# Autodesk Inventor assembly: !Ramp
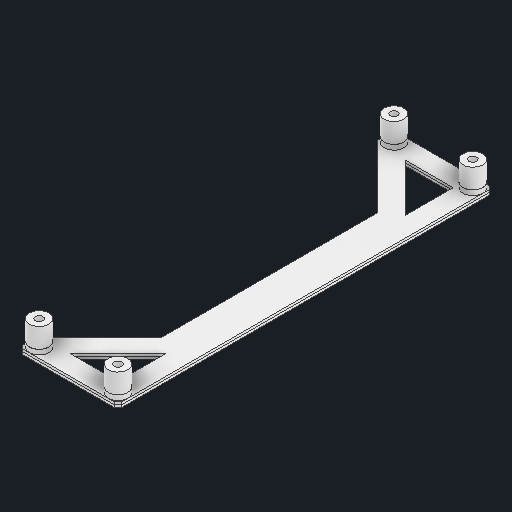
[picture p0: Inventor's stored thumbnail of the model, 512x512]
Saved by Autodesk Inventor 2025 (Build 290162000, 162)
## iProperties
Created: 2024-12-22
Part Number: !Ramp
Document SubType Name: Assembly
Designer: Averey Ku
Author: Averey Ku
## Documents named in this file (5)
- D:\VEX\High Stakes\CAD\V4\Chassis\Ramp\!Ramp.iam
- D:\VEX\High Stakes\CAD\V4\Chassis\Ramp\Custom Parts\Ramp.ipt
- D:\VEX\High Stakes\CAD\ROBOPROS-CAD-Inventor\Motion\Spacers\Spacer Nylon .500 OD.ipt
- D:\VEX\High Stakes\CAD\ROBOPROS-CAD-Inventor\Motion\Spacers\Spacer Nylon .500 OD\NSpacer White .500 OD x .500.ipt
- D:\VEX\High Stakes\CAD\ROBOPROS-CAD-Inventor\Motion\Spacers\Spacer Nylon .500 OD\NSpacer White .500 OD x .125.ipt
## Components (10 placed, 3 different names)
1. Ramp:1 — Insert:3, Insert:5, Insert:7, Insert:8, Insert:11, Mate:1
2. NSpacer White .500 OD x .500:2 — Insert:6
3. NSpacer White .500 OD x .500:4 — Insert:4
4. NSpacer White .500 OD x .500:6 — Insert:10
5. NSpacer White .500 OD x .500:8 — Insert:9
6. NSpacer White .500 OD x .125:9 — Insert:5, Insert:6
7. NSpacer White .500 OD x .125:10 — Insert:3, Insert:4
8. NSpacer White .500 OD x .125:11 — Insert:7, Insert:9
9. NSpacer White .500 OD x .125:12 — Insert:8, Insert:10
10. Ramp:2 — Insert:11, Mate:1
## Relationships (10: Insert 9, Mate 1)
- Insert:3: Ramp:1 ↔ NSpacer White .500 OD x .125:10
- Insert:4: NSpacer White .500 OD x .500:4 ↔ NSpacer White .500 OD x .125:10
- Insert:5: Ramp:1 ↔ NSpacer White .500 OD x .125:9
- Insert:6: NSpacer White .500 OD x .500:2 ↔ NSpacer White .500 OD x .125:9
- Insert:7: Ramp:1 ↔ NSpacer White .500 OD x .125:11
- Insert:8: Ramp:1 ↔ NSpacer White .500 OD x .125:12
- Insert:9: NSpacer White .500 OD x .500:8 ↔ NSpacer White .500 OD x .125:11
- Insert:10: NSpacer White .500 OD x .500:6 ↔ NSpacer White .500 OD x .125:12
- Insert:11: Ramp:1 ↔ Ramp:2
- Mate:1: Ramp:1 ↔ Ramp:2
